# Autodesk Inventor assembly: MainAssy_MIR1
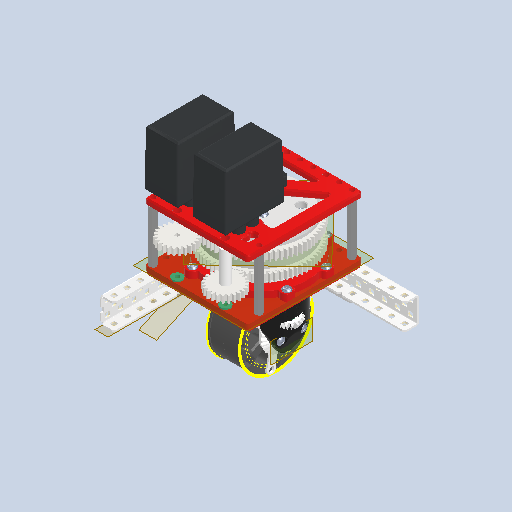
[picture p0: Inventor's stored thumbnail of the model, 512x512]
Saved by Autodesk Inventor 2023 (Build 270158000, 158)
## iProperties
Created: 2022-10-29
Part Number: MainAssy_MIR1
Document SubType Name: Assembly
Designer: zac-h
Author: zac-h
## Documents named in this file (41)
- C:\Users\Zac Hah\Documents\GitHub\spin-up-cad\guardSwerve5\MainAssy_MIR1.iam
- C:\Users\Zac Hah\Documents\GitHub\spin-up-cad\guardSwerve5\WheelHalf_MIR2.ipt
- C:\Users\Zac Hah\Documents\GitHub\spin-up-cad\guardSwerve5\WheelHalf_MIR_MIR1.ipt
- C:\Users\Zac Hah\Documents\GitHub\spin-up-cad\guardSwerve5\Carriage_MIR1.ipt
- C:\Users\Zac Hah\Documents\GitHub\spin-up-cad\guardSwerve5\MainAssy\Design Accelerator\Bevel Gears1_MIR1.iam
- C:\Users\Zac Hah\Documents\GitHub\spin-up-cad\VEX-CAD-Inventor-1.3.0\VEX-CAD-Inventor-1.3.0\Motion\Circle Insert_MIR1.ipt
- C:\Users\Zac Hah\Documents\GitHub\spin-up-cad\VEX-CAD-Inventor-1.3.0\VEX-CAD-Inventor-1.3.0\Structure\Hardware\Screw Steel - Star\SScrew Star Smooth .250.ipt
- C:\Users\zac-h\Documents\CAD\VEX-CAD-Inventor-1.3.0\VEX-CAD-Inventor-1.3.0\Structure\Hardware\Screw Steel - Star.ipt
- C:\Users\Zac Hah\Documents\GitHub\spin-up-cad\guardSwerve5\Baseplate_MIR1.ipt
- C:\Users\Zac Hah\Documents\GitHub\spin-up-cad\VEX-CAD-Inventor-1.3.0\VEX-CAD-Inventor-1.3.0\Structure\C-Channels\Aluminum 1x2x1\Alu C 1x2x1x10_MIR1.ipt
- C:\Users\Zac Hah\Documents\GitHub\spin-up-cad\guardSwerve5\UpperRaceRing_MIR1.ipt
- C:\Users\Zac Hah\Documents\GitHub\spin-up-cad\guardSwerve1\bearingsleeve_MIR3.ipt
- C:\Users\Zac Hah\Documents\GitHub\spin-up-cad\guardSwerve5\608bearing_MIR1.ipt
- C:\Users\Zac Hah\Documents\GitHub\spin-up-cad\guardSwerve5\SteeringCoupler_MIR1.ipt
- C:\Users\Zac Hah\Documents\GitHub\spin-up-cad\guardSwerve5\MainAssy\Design Accelerator\Spur Gears1_MIR1.iam
- C:\Users\Zac Hah\Documents\GitHub\spin-up-cad\guardSwerve5\MainAssy\Design Accelerator\Spur Gears2_MIR1.iam
- C:\Users\Zac Hah\Documents\GitHub\spin-up-cad\guardSwerve5\MainAssy\Design Accelerator\Spur Gears4_MIR1.iam
- C:\Users\Zac Hah\Documents\GitHub\spin-up-cad\guardSwerve5\MainAssy\Design Accelerator\Spur Gears5_MIR1.iam
- C:\Users\Zac Hah\Documents\GitHub\spin-up-cad\VEX-CAD-Inventor-1.3.0\VEX-CAD-Inventor-1.3.0\Structure\Hardware\Screw Steel - Star\SScrew Star Smooth .500.ipt
- C:\Users\Zac Hah\Documents\GitHub\spin-up-cad\guardSwerve5\MainAssy\Design Accelerator\Spur Gears3_MIR1.iam
- C:\Users\Zac Hah\Documents\GitHub\spin-up-cad\guardSwerve5\MainAssy\Design Accelerator\Spur Gears6_MIR1.iam
- C:\Users\Zac Hah\Documents\GitHub\spin-up-cad\guardSwerve5\UpperRingSeat_MIR1.ipt
- C:\Users\Zac Hah\Documents\GitHub\spin-up-cad\VEX-CAD-Inventor-1.3.0\VEX-CAD-Inventor-1.3.0\Structure\Hardware\Screw Steel - Star\SScrew Star Smooth 1.000.ipt
- C:\Users\Zac Hah\Documents\GitHub\spin-up-cad\guardSwerve5\DiffCap_MIR1.ipt
- C:\Users\Zac Hah\Documents\GitHub\spin-up-cad\VEX-CAD-Inventor-1.3.0\VEX-CAD-Inventor-1.3.0\Motion\Square Insert_MIR1.ipt
- C:\Users\Zac Hah\Documents\GitHub\spin-up-cad\VEX-CAD-Inventor-1.3.0\VEX-CAD-Inventor-1.3.0\Structure\Hardware\Screw Steel - Star\SScrew Star Smooth .875.ipt
- C:\Users\Zac Hah\Documents\GitHub\spin-up-cad\VEX-CAD-Inventor-1.3.0\VEX-CAD-Inventor-1.3.0\Structure\Hardware\Nut Nylock_MIR3.ipt
- C:\Users\Zac Hah\Documents\GitHub\spin-up-cad\VEX-CAD-Inventor-1.3.0\VEX-CAD-Inventor-1.3.0\Structure\Hardware\Screw Steel - Star\SScrew Star Smooth 1.250.ipt
- C:\Users\Zac Hah\Documents\GitHub\spin-up-cad\VEX-CAD-Inventor-1.3.0\VEX-CAD-Inventor-1.3.0\Motion\Shaft LS\Shaft LS 3.0 in.ipt
- C:\Users\zac-h\Documents\CAD\VEX-CAD-Inventor-1.3.0\VEX-CAD-Inventor-1.3.0\Motion\Shaft LS.ipt
- C:\Users\Zac Hah\Documents\GitHub\spin-up-cad\VEX-CAD-Inventor-1.3.0\VEX-CAD-Inventor-1.3.0\Structure\Hardware\Screw Steel - Star\SScrew Star Smooth 1.750.ipt
- C:\Users\Zac Hah\Documents\GitHub\spin-up-cad\VEX-CAD-Inventor-1.3.0\VEX-CAD-Inventor-1.3.0\Structure\Standoff\Standoff 2.00.ipt
- C:\Users\zac-h\Documents\CAD\VEX-CAD-Inventor-1.3.0\VEX-CAD-Inventor-1.3.0\Structure\Standoff.ipt
- C:\Users\Zac Hah\Documents\GitHub\spin-up-cad\guardSwerve5\TopPlate_MIR1.ipt
- C:\Users\Zac Hah\Documents\GitHub\spin-up-cad\VEX-CAD-Inventor-1.3.0\VEX-CAD-Inventor-1.3.0\Electronics\V5 Simple Motor_MIR3.ipt
- C:\Users\Zac Hah\Documents\GitHub\spin-up-cad\VEX-CAD-Inventor-1.3.0\VEX-CAD-Inventor-1.3.0\Electronics\Sensors\Potentiometer V2_MIR1.ipt
- C:\Users\Zac Hah\Documents\GitHub\spin-up-cad\VEX-CAD-Inventor-1.3.0\VEX-CAD-Inventor-1.3.0\Structure\Hardware\Screw Steel - Star\SScrew Star Smooth .750.ipt
- C:\Users\Zac Hah\Documents\GitHub\spin-up-cad\guardSwerve5\UnderGusset_MIR1.ipt
- C:\Users\Zac Hah\Documents\GitHub\spin-up-cad\VEX-CAD-Inventor-1.3.0\VEX-CAD-Inventor-1.3.0\Structure\Standoff\Standoff 1.00.ipt
- C:\Users\Zac Hah\Documents\GitHub\spin-up-cad\guardSwerve5\1.2inSpacer_MIR1.ipt
- C:\Users\Zac Hah\Documents\GitHub\spin-up-cad\VEX-CAD-Inventor-1.3.0\VEX-CAD-Inventor-1.3.0\Motion\0.188 ID x 0.500 OD x 0.196 WD (Radial Bearing) (217-3246).step
## Components (84 placed, 36 different names)
1. WheelHalf_MIR2:1 — Mate:1
2. WheelHalf_MIR_MIR1:1 — Flush:1, Angle:5, Mate:25
3. Carriage_MIR1:1 — Flush:1, Angle:4, Mate:24, Mate:4, Mate:7, Mate:6, Mate:5, Insert:3, Insert:11, Insert:12, Flush:2, Insert:39, Insert:38, Insert:37, Insert:36
4. Bevel Gears1_MIR1:1 [sub-assembly] — Angle:5, Mate:25, Angle:4, Mate:24, Mate:4, Mate:1
5. Circle Insert_MIR1:1 — Mate:7, Mate:6, Mate:5
6. Circle Insert_MIR1:2 — Insert:49
7. Circle Insert_MIR1:3 — Insert:44
8. Baseplate_MIR1:1 — Flush:2, Insert:21, Insert:14, Insert:16, Insert:15, Flush:4, Flush:3, Insert:28, Insert:27, Insert:69, Insert:66, Insert:67, Insert:68
9. Alu C 1x2x1x10_MIR1:1 — Insert:21, Insert:14, Flush:14, Flush:13
10. Alu C 1x2x1x10_MIR1:2 — Insert:16, Insert:15
11. UpperRaceRing_MIR1:1 — Flush:4, Flush:3, Insert:29
12. SteeringCoupler_MIR1:1 — Flush:5, Insert:31, Mate:21, Mate:20, Insert:32, Insert:33, Insert:34, Flush:8, Insert:45, Insert:63, Insert:64, Insert:65
13. Spur Gears1_MIR1:1 [sub-assembly] — Insert:49, Insert:31, Flush:7
14. Spur Gears2_MIR1:1 [sub-assembly] — Mate:21, Mate:20, Flush:11, Mate:23, Insert:30
15. Spur Gears4_MIR1:1 [sub-assembly] — Flush:11, Mate:23, Insert:30
16. Circle Insert_MIR1:4 — Insert:28, Insert:85
17. Circle Insert_MIR1:5 — Insert:27, Mate:15
18. Spur Gears5_MIR1:1 [sub-assembly] — Flush:7, Mate:15, Flush:15
19. Spur Gears3_MIR1:1 [sub-assembly] — Insert:32, Insert:43
20. Spur Gears3_MIR1:2 [sub-assembly] — Insert:44, Insert:33
21. Spur Gears6_MIR1:1 [sub-assembly] — Insert:34, Insert:42
22. UpperRingSeat_MIR1:1 — Flush:8, Insert:35, Flush:10, Flush:9, Insert:48
23. Spur Gears1_MIR1:2 [sub-assembly] — Insert:35, Insert:51
24. SScrew Star Smooth 1.000:4 — Insert:39
25. SScrew Star Smooth 1.000:5 — Insert:38
26. SScrew Star Smooth 1.000:6 — Insert:37
27. SScrew Star Smooth 1.000:7 — Insert:36
28. Spur Gears4_MIR1:2 [sub-assembly]
29. DiffCap_MIR1:1 — Flush:10, Flush:9, Insert:62, Insert:61, Insert:60
30. Square Insert_MIR1:1 — Insert:42
31. Circle Insert_MIR1:6 — Insert:43
32. SScrew Star Smooth .875:8 — Insert:45
33. Nut Nylock_MIR3:1 — Insert:48
34. Circle Insert_MIR1:7 — Insert:51
35. Shaft LS 3.0 in:1
36. SScrew Star Smooth 1.750:10 — Insert:62
37. SScrew Star Smooth 1.750:11 — Insert:61
38. SScrew Star Smooth 1.750:12 — Insert:60
39. Nut Nylock_MIR3:2 — Insert:63
40. Nut Nylock_MIR3:3 — Insert:64
41. Nut Nylock_MIR3:4 — Insert:65
42. Standoff 2.00:1 — Insert:69
43. Standoff 2.00:2 — Insert:66
44. Standoff 2.00:3 — Insert:67
45. Standoff 2.00:4 — Insert:68, Flush:12
46. TopPlate_MIR1:1 — Flush:12, Insert:73, Insert:72, Insert:71, Insert:70, Insert:80, Insert:77, Insert:78, Insert:79
47. V5 Simple Motor_MIR3:1 — Insert:73, Insert:72
48. V5 Simple Motor_MIR3:2 — Insert:71, Insert:70
49. Potentiometer V2_MIR1:1 — Insert:80, Insert:81, Insert:82
50. SScrew Star Smooth .750:13
51. SScrew Star Smooth .750:14 — Insert:77
52. SScrew Star Smooth .750:15 — Insert:78
53. SScrew Star Smooth .750:16 — Insert:79
54. SScrew Star Smooth .500:17 — Insert:81
55. SScrew Star Smooth .500:18 — Insert:82
56. UnderGusset_MIR1:1 — Flush:14, Flush:13, Insert:83, Insert:84
57. Standoff 1.00:5 — Insert:83
58. SScrew Star Smooth .500:19 — Insert:84
59. 1.2inSpacer_MIR1:1 — Flush:15
60. Spur Gears5_MIR1:2 [sub-assembly] — Insert:85
61. bearingsleeve_MIR3:1 — Insert:3, Insert:2
62. 608bearing_MIR1:1 — Insert:2, Flush:5
63. bearingsleeve_MIR3:2
64. 608bearing_MIR1:2
65. bearingsleeve_MIR3:3
66. 608bearing_MIR1:3
67. bearingsleeve_MIR3:4
68. 608bearing_MIR1:4
69. SScrew Star Smooth .250:1 — Insert:11
70. SScrew Star Smooth .250:2 — Insert:12
71. SScrew Star Smooth .250:20
72. SScrew Star Smooth .250:21
73. SScrew Star Smooth .500:3 — Insert:29
74. SScrew Star Smooth .500:22
75. SScrew Star Smooth .500:23
76. SScrew Star Smooth .500:24
77. SScrew Star Smooth .500:25
78. SScrew Star Smooth .500:26
79. SScrew Star Smooth .500:27
80. SScrew Star Smooth .500:28
81. SScrew Star Smooth 1.250:9
82. SScrew Star Smooth 1.250:29
83. SScrew Star Smooth 1.250:30
84. SScrew Star Smooth 1.250:31
## Component patterns: (4 elements, first: bearingsleeve_MIR3:1 + 608bearing_MIR1:1), (2 elements, first: SScrew Star Smooth .250:1 + SScrew Star Smooth .250:2), (8 elements, first: SScrew Star Smooth .500:3), (4 elements, first: SScrew Star Smooth 1.250:9)
## Relationships (78: Insert 51, Mate 23, Angle 2, Flush 2)
- Flush:1 [Mate]: WheelHalf_MIR_MIR1:1 ↔ Carriage_MIR1:1
- Angle:5 (0 deg): WheelHalf_MIR_MIR1:1 ↔ Bevel Gears1_MIR1:1
- Mate:25: WheelHalf_MIR_MIR1:1 ↔ Bevel Gears1_MIR1:1
- Angle:4 (0 deg): Carriage_MIR1:1 ↔ Bevel Gears1_MIR1:1
- Mate:24: Carriage_MIR1:1 ↔ Bevel Gears1_MIR1:1
- Mate:4: Carriage_MIR1:1 ↔ Bevel Gears1_MIR1:1
- Mate:1: WheelHalf_MIR2:1 ↔ Bevel Gears1_MIR1:1
- Mate:7: Carriage_MIR1:1 ↔ Circle Insert_MIR1:1
- Mate:6: Carriage_MIR1:1 ↔ Circle Insert_MIR1:1
- Mate:5: Carriage_MIR1:1 ↔ Circle Insert_MIR1:1
- Insert:3: Carriage_MIR1:1 ↔ bearingsleeve_MIR3:1
- Insert:2: bearingsleeve_MIR3:1 ↔ 608bearing_MIR1:1
- Insert:11: Carriage_MIR1:1 ↔ SScrew Star Smooth .250:1
- Insert:12: Carriage_MIR1:1 ↔ SScrew Star Smooth .250:2
- Flush:2 [Mate]: Carriage_MIR1:1 ↔ Baseplate_MIR1:1
- Insert:21: Baseplate_MIR1:1 ↔ Alu C 1x2x1x10_MIR1:1
- Insert:14: Baseplate_MIR1:1 ↔ Alu C 1x2x1x10_MIR1:1
- Insert:16: Baseplate_MIR1:1 ↔ Alu C 1x2x1x10_MIR1:2
- Insert:15: Baseplate_MIR1:1 ↔ Alu C 1x2x1x10_MIR1:2
- Flush:4 [Mate]: Baseplate_MIR1:1 ↔ UpperRaceRing_MIR1:1
- Flush:3 [Mate]: Baseplate_MIR1:1 ↔ UpperRaceRing_MIR1:1
- Flush:5 [Mate]: SteeringCoupler_MIR1:1 ↔ 608bearing_MIR1:1
- Insert:49: Circle Insert_MIR1:2 ↔ Spur Gears1_MIR1:1
- Insert:31: SteeringCoupler_MIR1:1 ↔ Spur Gears1_MIR1:1
- Mate:21: SteeringCoupler_MIR1:1 ↔ Spur Gears2_MIR1:1
- Mate:20: SteeringCoupler_MIR1:1 ↔ Spur Gears2_MIR1:1
- Flush:11: Spur Gears2_MIR1:1 ↔ Spur Gears4_MIR1:1
- Mate:23: Spur Gears2_MIR1:1 ↔ Spur Gears4_MIR1:1
- Insert:30: Spur Gears2_MIR1:1 ↔ Spur Gears4_MIR1:1
- Insert:29: UpperRaceRing_MIR1:1 ↔ SScrew Star Smooth .500:3
- Insert:28: Baseplate_MIR1:1 ↔ Circle Insert_MIR1:4
- Insert:27: Baseplate_MIR1:1 ↔ Circle Insert_MIR1:5
- Flush:7: Spur Gears1_MIR1:1 ↔ Spur Gears5_MIR1:1
- Mate:15: Circle Insert_MIR1:5 ↔ Spur Gears5_MIR1:1
- Insert:32: SteeringCoupler_MIR1:1 ↔ Spur Gears3_MIR1:1
- Insert:44: Circle Insert_MIR1:3 ↔ Spur Gears3_MIR1:2
- Insert:33: SteeringCoupler_MIR1:1 ↔ Spur Gears3_MIR1:2
- Insert:34 (1.27 mm): SteeringCoupler_MIR1:1 ↔ Spur Gears6_MIR1:1
- Flush:8 [Mate]: SteeringCoupler_MIR1:1 ↔ UpperRingSeat_MIR1:1
- Insert:35: UpperRingSeat_MIR1:1 ↔ Spur Gears1_MIR1:2
- Insert:39: Carriage_MIR1:1 ↔ SScrew Star Smooth 1.000:4
- Insert:38: Carriage_MIR1:1 ↔ SScrew Star Smooth 1.000:5
- Insert:37: Carriage_MIR1:1 ↔ SScrew Star Smooth 1.000:6
- Insert:36: Carriage_MIR1:1 ↔ SScrew Star Smooth 1.000:7
- Flush:10 [Mate]: UpperRingSeat_MIR1:1 ↔ DiffCap_MIR1:1
- Flush:9 [Mate]: UpperRingSeat_MIR1:1 ↔ DiffCap_MIR1:1
- Insert:42: Spur Gears6_MIR1:1 ↔ Square Insert_MIR1:1
- Insert:43: Spur Gears3_MIR1:1 ↔ Circle Insert_MIR1:6
- Insert:45: SteeringCoupler_MIR1:1 ↔ SScrew Star Smooth .875:8
- Insert:48: UpperRingSeat_MIR1:1 ↔ Nut Nylock_MIR3:1
- Insert:51: Spur Gears1_MIR1:2 ↔ Circle Insert_MIR1:7
- Insert:62: DiffCap_MIR1:1 ↔ SScrew Star Smooth 1.750:10
- Insert:61: DiffCap_MIR1:1 ↔ SScrew Star Smooth 1.750:11
- Insert:60: DiffCap_MIR1:1 ↔ SScrew Star Smooth 1.750:12
- Insert:63: SteeringCoupler_MIR1:1 ↔ Nut Nylock_MIR3:2
- Insert:64: SteeringCoupler_MIR1:1 ↔ Nut Nylock_MIR3:3
- Insert:65: SteeringCoupler_MIR1:1 ↔ Nut Nylock_MIR3:4
- Insert:69: Baseplate_MIR1:1 ↔ Standoff 2.00:1
- Insert:66: Baseplate_MIR1:1 ↔ Standoff 2.00:2
- Insert:67: Baseplate_MIR1:1 ↔ Standoff 2.00:3
- Insert:68: Baseplate_MIR1:1 ↔ Standoff 2.00:4
- Flush:12 [Mate]: Standoff 2.00:4 ↔ TopPlate_MIR1:1
- Insert:73: TopPlate_MIR1:1 ↔ V5 Simple Motor_MIR3:1
- Insert:72: TopPlate_MIR1:1 ↔ V5 Simple Motor_MIR3:1
- Insert:71: TopPlate_MIR1:1 ↔ V5 Simple Motor_MIR3:2
- Insert:70: TopPlate_MIR1:1 ↔ V5 Simple Motor_MIR3:2
- Insert:80: TopPlate_MIR1:1 ↔ Potentiometer V2_MIR1:1
- Insert:77: TopPlate_MIR1:1 ↔ SScrew Star Smooth .750:14
- Insert:78: TopPlate_MIR1:1 ↔ SScrew Star Smooth .750:15
- Insert:79: TopPlate_MIR1:1 ↔ SScrew Star Smooth .750:16
- Insert:81: Potentiometer V2_MIR1:1 ↔ SScrew Star Smooth .500:17
- Insert:82: Potentiometer V2_MIR1:1 ↔ SScrew Star Smooth .500:18
- Flush:14 [Mate]: Alu C 1x2x1x10_MIR1:1 ↔ UnderGusset_MIR1:1
- Flush:13 [Mate]: Alu C 1x2x1x10_MIR1:1 ↔ UnderGusset_MIR1:1
- Insert:83: UnderGusset_MIR1:1 ↔ Standoff 1.00:5
- Insert:84: UnderGusset_MIR1:1 ↔ SScrew Star Smooth .500:19
- Flush:15 [Mate]: Spur Gears5_MIR1:1 ↔ 1.2inSpacer_MIR1:1
- Insert:85 (28.575 mm): Circle Insert_MIR1:4 ↔ Spur Gears5_MIR1:2
